# Autodesk Inventor assembly: Knee
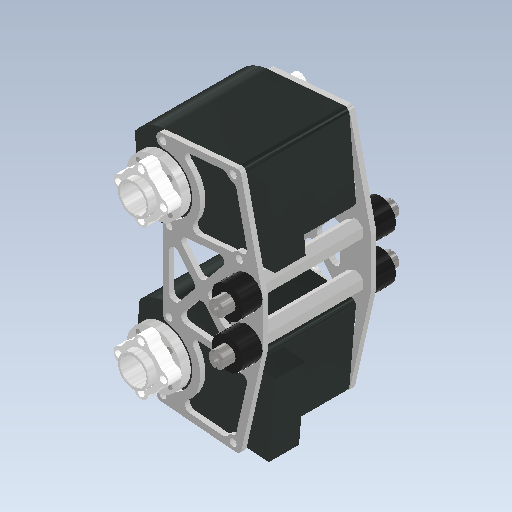
[picture p0: Inventor's stored thumbnail of the model, 512x512]
Saved by Autodesk Inventor 2020.4 (Build 244396000, 396)
## iProperties
Created: 2021-09-06
Part Number: Knee
Document SubType Name: Assembly
Designer: Masato
Mass: 264.861 g
Surface Area: 473.637 cm^2
Volume: 130.531 cm^3
Density: 2.0291 g/cm^3
Author: Masato
## Documents named in this file (11)
- C:\Users\masato\Documents\Inventor\CITBrains\OpenPlatform_ver3_0\LowerBody\Knee\Knee.iam
- C:\Users\masato\Documents\Inventor\CITBrains\OpenPlatform_ver3_0\LowerBody\Knee\Knee_side_frame.ipt
- C:\Users\masato\Documents\Inventor\CITBrains\OpenPlatform_ver3_0\Ready_Made\B3M11xx.ipt
- C:\Users\masato\Documents\Inventor\CITBrains\OpenPlatform_ver3_0\LowerBody\Link\Knee_clamp.ipt
- C:\Users\masato\Documents\Inventor\CITBrains\OpenPlatform_ver3_0\Ready_Made\free_horn.ipt
- C:\Users\masato\Documents\Inventor\CITBrains\OpenPlatform_ver3_0\Ready_Made\SLSBF6-39_5-M3-N3.ipt
- C:\Users\masato\Documents\Inventor\CITBrains\OpenPlatform_ver3_0\Ready_Made\UUW-0312-10BH.ipt
- C:\Users\masato\Documents\Inventor\CITBrains\OpenPlatform_ver3_0\Ready_Made\WSSS-12-10-8.ipt
- C:\Users\masato\Documents\Inventor\CITBrains\OpenPlatform_ver3_0\Ready_Made\CC-0612-25B.ipt
- C:\Users\masato\Documents\Inventor\CITBrains\OpenPlatform_ver3_0\Ready_Made\CC-0612-20B.ipt
- C:\Users\masato\Documents\Inventor\CITBrains\OpenPlatform_ver3_0\Ready_Made\BRU-311S.ipt
## Components (36 placed, 10 different names)
1. Knee_side_frame:1 — 挿入:1, 挿入:2, 挿入:3, 挿入:4, 挿入:5, 挿入:6, 挿入:7, 挿入:8, メイト:1, 挿入:41, 挿入:42, 挿入:45, 挿入:46
2. Knee_side_frame:2 — 挿入:9, 挿入:10, 挿入:11, 挿入:12, 挿入:13, 挿入:14, 挿入:15, 挿入:16, 挿入:43, 挿入:44, 挿入:47, 挿入:48
3. B3M11xx:1 — 挿入:1, 挿入:2, 挿入:5, 挿入:6, 挿入:9, 挿入:10, 挿入:15, 挿入:16, 挿入:31, 挿入:33
4. B3M11xx:2 — 挿入:3, 挿入:4, 挿入:7, 挿入:8, 挿入:11, 挿入:12, 挿入:13, 挿入:14, 挿入:32, 挿入:34
5. Knee_clamp:1 — 挿入:32, 挿入:61
6. Knee_clamp:2 — 挿入:31, 挿入:62
7. Knee_clamp:3 — 挿入:36, 挿入:63
8. Knee_clamp:4 — 挿入:35, 挿入:64
9. free_horn:1 — 挿入:33, 挿入:35
10. free_horn:2 — 挿入:34, 挿入:36
11. SLSBF6-39_5-M3-N3:1 — 挿入:41, 挿入:43
12. SLSBF6-39_5-M3-N3:2 — 挿入:42, 挿入:44
13. UUW-0312-10BH:1 — 挿入:45, 挿入:65, 挿入:77
14. UUW-0312-10BH:2 — 挿入:46, 挿入:66, 挿入:78
15. UUW-0312-10BH:3 — 挿入:47, 挿入:67, 挿入:79
16. UUW-0312-10BH:4 — 挿入:48, 挿入:68, 挿入:80
17. WSSS-12-10-8:1 — 挿入:64
18. WSSS-12-10-8:2 — 挿入:63
19. WSSS-12-10-8:3 — 挿入:62
20. WSSS-12-10-8:4 — 挿入:61
21. CC-0612-25B:1 — 挿入:66, 挿入:70
22. CC-0612-25B:2 — 挿入:65, 挿入:69
23. CC-0612-25B:3 — 挿入:67, 挿入:72
24. CC-0612-25B:4 — 挿入:68, 挿入:71
25. CC-0612-20B:1 — 挿入:69, 挿入:75
26. CC-0612-20B:2 — 挿入:70, 挿入:76
27. CC-0612-20B:3 — 挿入:71, 挿入:74
28. CC-0612-20B:4 — 挿入:72, 挿入:73
29. CC-0612-20B:5 — 挿入:75
30. CC-0612-20B:6 — 挿入:76
31. CC-0612-20B:7 — 挿入:73
32. CC-0612-20B:8 — 挿入:74
33. BRU-311S:1 — 挿入:77
34. BRU-311S:2 — 挿入:78
35. BRU-311S:3 — 挿入:80
36. BRU-311S:4 — 挿入:79
## Relationships (51: Insert 50, Mate 1)
- 挿入:1 [Insert]: Knee_side_frame:1 ↔ B3M11xx:1
- 挿入:2 [Insert]: Knee_side_frame:1 ↔ B3M11xx:1
- 挿入:3 [Insert]: Knee_side_frame:1 ↔ B3M11xx:2
- 挿入:4 [Insert]: Knee_side_frame:1 ↔ B3M11xx:2
- 挿入:5 [Insert]: Knee_side_frame:1 ↔ B3M11xx:1
- 挿入:6 [Insert]: Knee_side_frame:1 ↔ B3M11xx:1
- 挿入:7 [Insert]: Knee_side_frame:1 ↔ B3M11xx:2
- 挿入:8 [Insert]: Knee_side_frame:1 ↔ B3M11xx:2
- 挿入:9 [Insert]: Knee_side_frame:2 ↔ B3M11xx:1
- 挿入:10 [Insert]: Knee_side_frame:2 ↔ B3M11xx:1
- 挿入:11 [Insert]: Knee_side_frame:2 ↔ B3M11xx:2
- 挿入:12 [Insert]: Knee_side_frame:2 ↔ B3M11xx:2
- 挿入:13 [Insert]: Knee_side_frame:2 ↔ B3M11xx:2
- 挿入:14 [Insert]: Knee_side_frame:2 ↔ B3M11xx:2
- 挿入:15 [Insert]: Knee_side_frame:2 ↔ B3M11xx:1
- 挿入:16 [Insert]: Knee_side_frame:2 ↔ B3M11xx:1
- 挿入:31 [Insert]: B3M11xx:1 ↔ Knee_clamp:2
- 挿入:32 [Insert]: B3M11xx:2 ↔ Knee_clamp:1
- 挿入:33 [Insert]: B3M11xx:1 ↔ free_horn:1
- 挿入:34 [Insert]: B3M11xx:2 ↔ free_horn:2
- 挿入:35 [Insert]: Knee_clamp:4 ↔ free_horn:1
- 挿入:36 [Insert]: Knee_clamp:3 ↔ free_horn:2
- メイト:1 [Mate] (19.75 mm): Knee_side_frame:1
- 挿入:41 [Insert]: Knee_side_frame:1 ↔ SLSBF6-39_5-M3-N3:1
- 挿入:42 [Insert]: Knee_side_frame:1 ↔ SLSBF6-39_5-M3-N3:2
- 挿入:43 [Insert]: Knee_side_frame:2 ↔ SLSBF6-39_5-M3-N3:1
- 挿入:44 [Insert]: Knee_side_frame:2 ↔ SLSBF6-39_5-M3-N3:2
- 挿入:45 [Insert]: Knee_side_frame:1 ↔ UUW-0312-10BH:1
- 挿入:46 [Insert]: Knee_side_frame:1 ↔ UUW-0312-10BH:2
- 挿入:47 [Insert]: Knee_side_frame:2 ↔ UUW-0312-10BH:3
- 挿入:48 [Insert]: Knee_side_frame:2 ↔ UUW-0312-10BH:4
- 挿入:61 [Insert]: Knee_clamp:1 ↔ WSSS-12-10-8:4
- 挿入:62 [Insert]: Knee_clamp:2 ↔ WSSS-12-10-8:3
- 挿入:63 [Insert]: Knee_clamp:3 ↔ WSSS-12-10-8:2
- 挿入:64 [Insert]: Knee_clamp:4 ↔ WSSS-12-10-8:1
- 挿入:65 [Insert]: UUW-0312-10BH:1 ↔ CC-0612-25B:2
- 挿入:66 [Insert]: UUW-0312-10BH:2 ↔ CC-0612-25B:1
- 挿入:67 [Insert]: UUW-0312-10BH:3 ↔ CC-0612-25B:3
- 挿入:68 [Insert]: UUW-0312-10BH:4 ↔ CC-0612-25B:4
- 挿入:69 [Insert]: CC-0612-25B:2 ↔ CC-0612-20B:1
- 挿入:70 [Insert]: CC-0612-25B:1 ↔ CC-0612-20B:2
- 挿入:71 [Insert]: CC-0612-25B:4 ↔ CC-0612-20B:3
- 挿入:72 [Insert]: CC-0612-25B:3 ↔ CC-0612-20B:4
- 挿入:73 [Insert]: CC-0612-20B:4 ↔ CC-0612-20B:7
- 挿入:74 [Insert]: CC-0612-20B:3 ↔ CC-0612-20B:8
- 挿入:75 [Insert]: CC-0612-20B:1 ↔ CC-0612-20B:5
- 挿入:76 [Insert]: CC-0612-20B:2 ↔ CC-0612-20B:6
- 挿入:77 [Insert]: UUW-0312-10BH:1 ↔ BRU-311S:1
- 挿入:78 [Insert]: UUW-0312-10BH:2 ↔ BRU-311S:2
- 挿入:79 [Insert]: UUW-0312-10BH:3 ↔ BRU-311S:4
- 挿入:80 [Insert]: UUW-0312-10BH:4 ↔ BRU-311S:3
